# Autodesk Inventor assembly: LZM-15ZT_rotameter_06-6_M3-H_Assembly
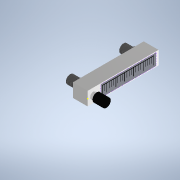
[picture p0: Inventor's stored thumbnail of the model, 180x180]
Saved by Autodesk Inventor 2020 (Build 240168000, 168)
## iProperties
Created: 2020-07-28
Part Number: LZM-15ZT_rotameter_06-6_M3-H_Assembly
Document SubType Name: Assembly
Designer: Samuel
Author: Samuel
## Documents named in this file (5)
- C:\Users\Samuel\Desktop\Rotameter\LZM-15ZT_rotameter_06-6_M3-H_Assembly.iam
- C:\Users\Samuel\Desktop\Rotameter\LZM-15ZT_rotameter_06-6_M3-H.ipt
- C:\Users\Samuel\Desktop\Rotameter\nut_din934_m6-10.ipt
- C:\Users\Samuel\Desktop\Rotameter\din m6-10 Flat point socket set screw.ipt
- C:\Users\Samuel\Desktop\Rotameter\din_6902-a_m6-200hv.ipt
## Components (7 placed, 4 different names)
1. LZM-15ZT_rotameter_06-6_M3-H:1 — Cylindrical:1, Cylindrical:2, Cylindrical:3, Cylindrical:4
2. nut_din934_m6-10:1 — Cylindrical:6
3. nut_din934_m6-10:2 — Cylindrical:5
4. din m6-10 Flat point socket set screw:1 — Cylindrical:2
5. din m6-10 Flat point socket set screw:2 — Cylindrical:1
6. din_6902-a_m6-200hv:1 — Cylindrical:3, Cylindrical:6
7. din_6902-a_m6-200hv:2 — Cylindrical:4, Cylindrical:5
## Relationships (6: CylindricalJoint 6)
- Cylindrical:1: LZM-15ZT_rotameter_06-6_M3-H:1 ↔ din m6-10 Flat point socket set screw:2
- Cylindrical:2: LZM-15ZT_rotameter_06-6_M3-H:1 ↔ din m6-10 Flat point socket set screw:1
- Cylindrical:3: LZM-15ZT_rotameter_06-6_M3-H:1 ↔ din_6902-a_m6-200hv:1
- Cylindrical:4: LZM-15ZT_rotameter_06-6_M3-H:1 ↔ din_6902-a_m6-200hv:2
- Cylindrical:5: nut_din934_m6-10:2 ↔ din_6902-a_m6-200hv:2
- Cylindrical:6: nut_din934_m6-10:1 ↔ din_6902-a_m6-200hv:1
